# Autodesk Inventor assembly: Shooting Mechanism Assembly
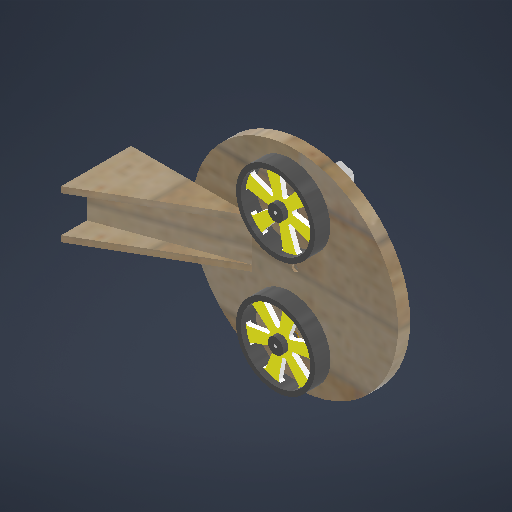
[picture p0: Inventor's stored thumbnail of the model, 512x512]
Saved by Autodesk Inventor 2026.2 (Build 302298000, 298)
## iProperties
Created: 2026-03-02
Part Number: Shooting Mechanism Assembly
Document SubType Name: Assembly
Designer: abdul
Author: abdul
## Documents named in this file (4)
- C:\Users\danda\OneDrive\Desktop\Basics Of Mecha\Project\Shooting Mechanism CAD\Shooting Mechanism Assembly.iam
- C:\Users\danda\OneDrive\Desktop\Basics Of Mecha\Project\Shooting Mechanism CAD\Base.ipt
- C:\Users\danda\OneDrive\Desktop\Basics Of Mecha\Project\Shooting Mechanism CAD\flywheel.ipt
- C:\Users\danda\OneDrive\Desktop\Basics Of Mecha\Project\Shooting Mechanism CAD\Dc Motor 3mm D Shaft.ipt
## Components (5 placed, 3 different names)
1. Base:1 — Mate:1, Mate:2, Mate:3, Mate:4
2. Dc Motor 3mm D Shaft:1 — Mate:1, Mate:4, Mate:9, Mate:11
3. Dc Motor 3mm D Shaft:2 — Mate:2, Mate:3, Mate:6, Mate:8, Mate:10
4. flywheel:2 — Mate:6, Mate:8, Mate:10
5. flywheel:3 — Mate:9, Mate:11
## Relationships (9: Mate 9)
- Mate:1: Base:1 ↔ Dc Motor 3mm D Shaft:1
- Mate:2: Base:1 ↔ Dc Motor 3mm D Shaft:2
- Mate:3: Base:1 ↔ Dc Motor 3mm D Shaft:2
- Mate:4: Base:1 ↔ Dc Motor 3mm D Shaft:1
- Mate:6: Dc Motor 3mm D Shaft:2 ↔ flywheel:2
- Mate:8: Dc Motor 3mm D Shaft:2 ↔ flywheel:2
- Mate:9: Dc Motor 3mm D Shaft:1 ↔ flywheel:3
- Mate:10: Dc Motor 3mm D Shaft:2 ↔ flywheel:2
- Mate:11: Dc Motor 3mm D Shaft:1 ↔ flywheel:3
